# Autodesk Inventor assembly: EBox
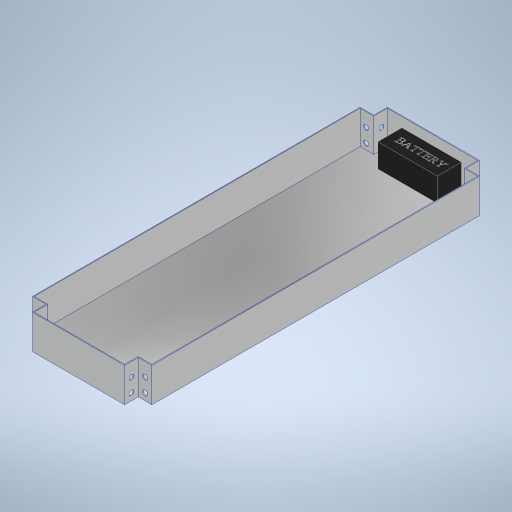
[picture p0: Inventor's stored thumbnail of the model, 512x512]
Saved by Autodesk Inventor 2023 (Build 270158000, 158)
## iProperties
Created: 2022-10-10
Part Number: EBox
Document SubType Name: Assembly
Designer: Nebil
Author: Nebil
## Documents named in this file (3)
- C:\Users\seene\Desktop\Stony Brook\SBRT\RoboRescue\GrabCAD\Robocup Rescue\Chassis\Electronics Box\EBox.iam
- C:\Users\seene\Desktop\Stony Brook\SBRT\RoboRescue\GrabCAD\Robocup Rescue\Chassis\Electronics Box\EBox-Parts\EBox-Frame.ipt
- C:\Users\seene\Desktop\Stony Brook\SBRT\RoboRescue\GrabCAD\Robocup Rescue\Chassis\Electronics Box\EBox-Parts\EBox-ArmBattery.ipt
## Components (2 placed, 2 different names)
1. EBox-Frame:1 — Mate:1, Mate:2
2. EBox-ArmBattery:1 — Mate:1, Mate:2
## Relationships (2: Mate 2)
- Mate:1: EBox-Frame:1 ↔ EBox-ArmBattery:1
- Mate:2: EBox-Frame:1 ↔ EBox-ArmBattery:1
